# Autodesk Inventor assembly: 15102898-16-A-0000
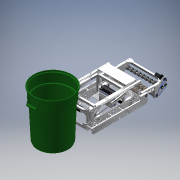
[picture p0: Inventor's stored thumbnail of the model, 180x180]
Saved by Autodesk Inventor 2017 (Build 210142000, 142)
## iProperties
Created: 2016-09-11
Part Number: 15102898-16-A-0000
Document SubType Name: Assembly
Designer: gus
Mass: 27886.1 g
Surface Area: 91797.7 cm^2
Volume: 21610.5 cm^3
Density: 1.2904 g/cm^3
Author: gus
## Documents named in this file (8)
- \\Mac\Home\Desktop\bunnybots 2016\15102898-16-Bunnybot-CAD\Bunnybot-To_be_renamed\15102898-16-A-0000\15102898-16-A-0000.iam
- \\Mac\Home\Desktop\bunnybots 2016\15102898-16-Bunnybot-CAD\Bunnybot-To_be_renamed\15102898-16-A-0000\15102898-16-A-0100\15102898-16-A-0100.iam
- \\Mac\Home\Desktop\bunnybots 2016\15102898-16-Bunnybot-CAD\Bunnybot-To_be_renamed\15102898-16-A-0000\15102898-16-A-0200\15102898-16-A-0200.iam
- \\Mac\Home\Desktop\bunnybots 2016\15102898-16-Bunnybot-CAD\Bunnybot-To_be_renamed\15102898-16-A-0000\15102898-16-A-0300\15102898-16-A-0300.iam
- \\Mac\Home\Desktop\bunnybots 2016\15102898-16-Bunnybot-CAD\Bunnybot-To_be_renamed\15102898-16-A-0000\recycling bin\RECYCLING_CAN.ipt
- \\Mac\Home\Desktop\bunnybots 2016\15102898-16-Bunnybot-CAD\Bunnybot-To_be_renamed\15102898-16-A-0000\15102898-16-A-0400\15102898-16-A-0400.iam
- \\Mac\Home\Desktop\bunnybots 2016\15102898-16-Bunnybot-CAD\Bunnybot-To_be_renamed\15102898-16-A-0000\15102898-16-A-0300\15102898-16-P-0306.ipt
- \\Mac\Home\Desktop\bunnybots 2016\15102898-16-Bunnybot-CAD\Bunnybot-To_be_renamed\15102898-16-A-0000\15102898-16-A-0300\15102898-16-P-0306_MIR.ipt
## Components (7 placed, 7 different names)
1. 15102898-16-A-0100:1 [sub-assembly] — Mate:1, Mate:3, Mate:4, Flush:1, Mate:5, Flush:2, Mate:6, Flush:3, Mate:7, Mate:8, Flush:5
2. 15102898-16-A-0200:1 [sub-assembly] — Mate:1, Mate:3, Mate:4
3. 15102898-16-A-0300:2 [sub-assembly] — Rotational:1
4. RECYCLING_CAN:1
5. 15102898-16-A-0400:1 [sub-assembly] — Mate:5, Flush:2, Mate:6
6. 15102898-16-P-0306:1 — Flush:3, Mate:7, Rotational:1, Mate:8, Flush:4, Flush:6
7. 15102898-16-P-0306_MIR:1 — Flush:4, Flush:5, Flush:6
## Relationships (14: Mate 7, Flush 6, RevoluteJoint 1)
- Mate:1: 15102898-16-A-0100:1 ↔ 15102898-16-A-0200:1
- Mate:3 (34.925 mm): 15102898-16-A-0100:1 ↔ 15102898-16-A-0200:1
- Mate:4 (3.175 mm): 15102898-16-A-0100:1 ↔ 15102898-16-A-0200:1
- Flush:1 (-291.973 mm): 15102898-16-A-0100:1
- Mate:5: 15102898-16-A-0100:1 ↔ 15102898-16-A-0400:1
- Flush:2: 15102898-16-A-0100:1 ↔ 15102898-16-A-0400:1
- Mate:6: 15102898-16-A-0100:1 ↔ 15102898-16-A-0400:1
- Flush:3: 15102898-16-A-0100:1 ↔ 15102898-16-P-0306:1
- Mate:7: 15102898-16-A-0100:1 ↔ 15102898-16-P-0306:1
- Rotational:1 [RevoluteJoint]: 15102898-16-A-0300:2 ↔ 15102898-16-P-0306:1
- Mate:8: 15102898-16-A-0100:1 ↔ 15102898-16-P-0306:1
- Flush:4: 15102898-16-P-0306:1 ↔ 15102898-16-P-0306_MIR:1
- Flush:5: 15102898-16-A-0100:1 ↔ 15102898-16-P-0306_MIR:1
- Flush:6: 15102898-16-P-0306:1 ↔ 15102898-16-P-0306_MIR:1
